# Autodesk Inventor assembly: EngineElectronics
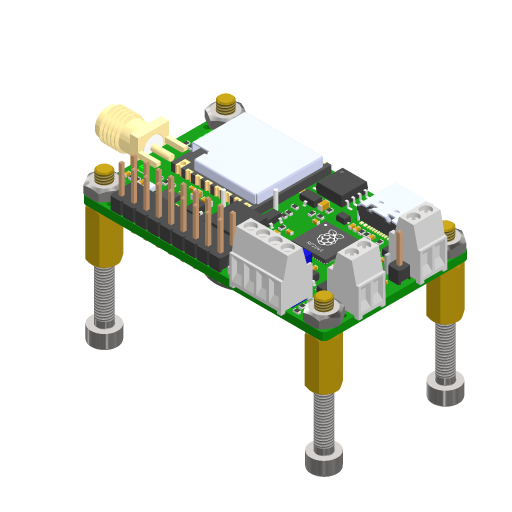
[picture p0: Inventor's stored thumbnail of the model, 512x512]
Saved by Autodesk Inventor 2024 (Build 280153000, 153)
## iProperties
Created: 2023-10-15
Part Number: EngineElectronics
Document SubType Name: Assembly
Designer: janwi
Author: janwi
## Documents named in this file (5)
- C:\Users\Jamie\Documents\Uni\DARE\PIP-IV-CAD-Files\Engine Section\Recovery\Electronics\EngineElectronics.iam
- C:\Users\Jamie\Documents\Uni\DARE\PIP-IV-CAD-Files\Payload Section\Electronics\M3_M_TO_F_10MM_STANDOFF.ipt
- C:\Users\Jamie\Documents\Uni\DARE\PIP-IV-CAD-Files\Content Centre Files\R2024\en-US\ISO 4762(2)\ISO 4762 - M3 x 16ISO.ipt
- C:\Users\Jamie\Documents\Uni\DARE\PIP-IV-CAD-Files\Payload Section\Electronics\Kolibri\Kolibri_rev1.1.iam
- C:\Users\Jamie\Documents\Uni\DARE\PIP-IV-CAD-Files\Content Centre Files\R2024\en-US\ISO 4032(1)\ISO 4032 - M3DIN EN.ipt
## Components (13 placed, 4 different names)
1. ISO 4762 M3 x 16:1
2. ISO 4762 M3 x 16:2
3. ISO 4762 M3 x 16:3
4. ISO 4762 M3 x 16:4
5. Kolibri_rev1.1:1 [sub-assembly] — Mate:3, Mate:4, Mate:5, Mate:7, Mate:9, Mate:11, Mate:13
6. DIN EN 24032 M3:1 — Mate:6, Mate:7
7. DIN EN 24032 M3:2 — Mate:8, Mate:9
8. DIN EN 24032 M3:3 — Mate:10, Mate:11
9. DIN EN 24032 M3:4 — Mate:12, Mate:13
10. M3_M_TO_F_10MM_STANDOFF:1 — Mate:8
11. M3_M_TO_F_10MM_STANDOFF:2 — Mate:4, Mate:5, Mate:6
12. M3_M_TO_F_10MM_STANDOFF:3 — Mate:10
13. M3_M_TO_F_10MM_STANDOFF:4 — Mate:3, Mate:12
## Component patterns: (4 elements, first: M3_M_TO_F_10MM_STANDOFF:1)
## Relationships (11: Mate 11)
- Mate:3: Kolibri_rev1.1:1 ↔ M3_M_TO_F_10MM_STANDOFF:4
- Mate:4: Kolibri_rev1.1:1 ↔ M3_M_TO_F_10MM_STANDOFF:2
- Mate:5: Kolibri_rev1.1:1 ↔ M3_M_TO_F_10MM_STANDOFF:2
- Mate:6: DIN EN 24032 M3:1 ↔ M3_M_TO_F_10MM_STANDOFF:2
- Mate:7: Kolibri_rev1.1:1 ↔ DIN EN 24032 M3:1
- Mate:8: DIN EN 24032 M3:2 ↔ M3_M_TO_F_10MM_STANDOFF:1
- Mate:9: Kolibri_rev1.1:1 ↔ DIN EN 24032 M3:2
- Mate:10: DIN EN 24032 M3:3 ↔ M3_M_TO_F_10MM_STANDOFF:3
- Mate:11: Kolibri_rev1.1:1 ↔ DIN EN 24032 M3:3
- Mate:12: DIN EN 24032 M3:4 ↔ M3_M_TO_F_10MM_STANDOFF:4
- Mate:13: Kolibri_rev1.1:1 ↔ DIN EN 24032 M3:4
